# Autodesk Inventor assembly: RoboAssembly
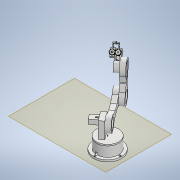
[picture p0: Inventor's stored thumbnail of the model, 180x180]
Saved by Autodesk Inventor 2022 (Build 260153000, 153)
## iProperties
Created: 2022-04-26
Part Number: RoboAssembly
Document SubType Name: Assembly
Designer: Adrian
Author: Adrian
## Documents named in this file (8)
- D:\Users\Adrian\Desktop\CAD for Physical Build\RoboAssembly.iam
- D:\Users\Adrian\Desktop\CAD for Physical Build\1stArm.ipt
- D:\Users\Adrian\Desktop\CAD for Physical Build\2ndArm.ipt
- D:\Users\Adrian\Desktop\CAD for Physical Build\Base top w servo housing.ipt
- D:\Users\Adrian\Desktop\CAD for Physical Build\Free gear.ipt
- D:\Users\Adrian\Desktop\CAD for Physical Build\NBase Part.ipt
- D:\Users\Adrian\Desktop\CAD for Physical Build\NeWConceptV2.0.ipt
- D:\Users\Adrian\Desktop\CAD for Physical Build\Servo new gear.ipt
## Components (7 placed, 7 different names)
1. BasePart — Mate:1, Insert:1
2. Base top w servo housing:1 — Insert:1, Insert:2
3. 1stArm:1 — Insert:2, Insert:3
4. 2ndArm:1 — Insert:3, Insert:4
5. EndEffectorBlock — Insert:4, Insert:5, Insert:6
6. Gripper1 — Insert:5, Rotation:1
7. Gripper2 — Insert:6, Rotation:1
## Relationships (8: Insert 6, Mate 1, RelateRotation 1)
- Mate:1: BasePart
- Insert:1: BasePart ↔ Base top w servo housing:1
- Insert:2: Base top w servo housing:1 ↔ 1stArm:1
- Insert:3: 1stArm:1 ↔ 2ndArm:1
- Insert:4: 2ndArm:1 ↔ EndEffectorBlock
- Insert:5 (-3 mm): EndEffectorBlock ↔ Gripper1
- Insert:6 (-7.4 mm): EndEffectorBlock ↔ Gripper2
- Rotation:1 [RelateRotation] (1 ul): Gripper1 ↔ Gripper2
